# Autodesk Inventor assembly: OuterShaftGear_v2
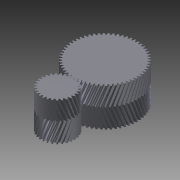
[picture p0: Inventor's stored thumbnail of the model, 180x180]
Saved by Autodesk Inventor 2014 SP1 (Build 180222100, 222)
## iProperties
Created: 2015-10-09
Part Number: OuterShaftGear_v2
Document SubType Name: Assembly
Designer: Sam
Author: Sam
## Documents named in this file (3)
- C:\Users\Sam\Documents\GitHub\Octanis1-CAD\CAD_Rover_Rev04_Musk\OuterShaftGear_v2.iam
- C:\Users\Sam\Documents\GitHub\Octanis1-CAD\CAD_Rover_Rev04_Musk\OuterShaftGear_v2\Design Accelerator\Spur Gears2.iam
- C:\Users\Sam\Documents\GitHub\Octanis1-CAD\CAD_Rover_Rev04_Musk\OuterShaftGear_v2\Design Accelerator\Spur Gears2_MIR3.iam
## Components (2 placed, 2 different names)
1. Spur Gears:2 [sub-assembly] — Rigid:1
2. Spur Gears2_MIR3:1 [sub-assembly] — Rigid:1
## Relationships (1: WeldJoint 1)
- Rigid:1 [WeldJoint]: Spur Gears:2 ↔ Spur Gears2_MIR3:1
